# Autodesk Inventor assembly: Assembly1
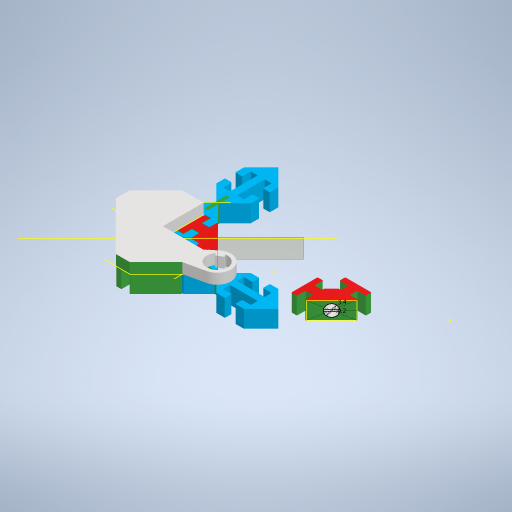
[picture p0: Inventor's stored thumbnail of the model, 512x512]
Saved by Autodesk Inventor 2023 (Build 270158000, 158)
## iProperties
Created: 2023-01-27
Part Number: Assembly1
Document SubType Name: Assembly
Designer: Asus
Author: Asus
## Documents named in this file (7)
- S:\Johannes\Uni\MetaMaterials\design\MetaSensingLight\Assembly1.iam
- S:\Johannes\Uni\MetaMaterials\design\MetaSensingLight\TmpPart1.ipt
- S:\Johannes\Uni\MetaMaterials\design\MetaSensingLight\TmpPart2.ipt
- S:\Johannes\Uni\MetaMaterials\design\MetaSensingLight\TmpPart3.ipt
- S:\Johannes\Uni\MetaMaterials\design\MetaSensingLight\TmpPart5.ipt
- S:\Johannes\Uni\MetaMaterials\design\MetaSensingLight\potHolderLeft.ipt
- S:\Johannes\Uni\MetaMaterials\design\MetaSensingLight\potHolderLeft2.ipt
## Components (8 placed, 6 different names)
1. TmpPart1:1 — Mate:1, Mate:2, Flush:2, Mate:3, Mate:4, Mate:5, Flush:3, Flush:4, Flush:8, Mate:8
2. TmpPart2:1
3. TmpPart3:1 — Flush:2, Mate:3, Mate:4
4. TmpPart5:1
5. potHolderLeft:1 — Mate:1, Mate:2
6. TmpPart1:2 — Mate:5, Flush:3, Flush:4, Mate:7, Mate:6, Flush:5, Flush:7, Flush:9
7. TmpPart2:2 — Mate:7, Mate:6, Flush:5
8. potHolderLeft2:1 — Flush:8, Mate:8, Flush:9
## Relationships (15: Mate 8, Flush 7)
- Mate:1 (0.2 mm): TmpPart1:1 ↔ potHolderLeft:1
- Mate:2 (0.2 mm): TmpPart1:1 ↔ potHolderLeft:1
- Flush:2: TmpPart1:1 ↔ TmpPart3:1
- Mate:3 (0.2 mm): TmpPart1:1 ↔ TmpPart3:1
- Mate:4 (0.2 mm): TmpPart1:1 ↔ TmpPart3:1
- Mate:5: TmpPart1:1 ↔ TmpPart1:2
- Flush:3: TmpPart1:1 ↔ TmpPart1:2
- Flush:4: TmpPart1:1 ↔ TmpPart1:2
- Mate:7: TmpPart1:2 ↔ TmpPart2:2
- Mate:6: TmpPart1:2 ↔ TmpPart2:2
- Flush:5: TmpPart1:2 ↔ TmpPart2:2
- Flush:7: TmpPart1:2
- Flush:8: TmpPart1:1 ↔ potHolderLeft2:1
- Mate:8: TmpPart1:1 ↔ potHolderLeft2:1
- Flush:9: TmpPart1:2 ↔ potHolderLeft2:1
